# Autodesk Inventor assembly: outerHorn slider
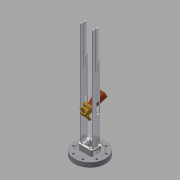
[picture p0: Inventor's stored thumbnail of the model, 180x180]
Saved by Autodesk Inventor 2015 SP1 (Build 190203100, 203)
## iProperties
Created: 2016-04-08
Part Number: outerHorn slider
Document SubType Name: Assembly
Designer: jad211
Author: jad211
## Documents named in this file (7)
- C:\ColdMatter\CADFiles\EDM Machine\Detection Region\Microwave Horn Assembly\outerHorn slider.iam
- C:\ColdMatter\CADFiles\EDM Machine\Detection Region\Microwave Horn Assembly\Horn with Flange.iam
- C:\ColdMatter\CADFiles\EDM Machine\Detection Region\Microwave Horn Assembly\Horn support.ipt
- C:\ColdMatter\CADFiles\EDM Machine\Pumping Region\coaxToWaveguidWG18.ipt
- C:\ColdMatter\CADFiles\EDM Machine\Detection Region\Microwave Horn Assembly\rod.ipt
- C:\ColdMatter\CADFiles\EDM Machine\Detection Region\Microwave Horn Assembly\DN63CF blank With Holes.ipt
- C:\ColdMatter\CADFiles\EDM Machine\Detection Region\Microwave Horn Assembly\supportHolder.ipt
## Components (10 placed, 6 different names)
1. Horn with Flange:1 [sub-assembly] — Mate:4, Mate:5, Flush:1, Mate:26, Mate:27, Mate:28, Mate:29, Mate:30, Mate:31, Mate:32
2. Horn support:1 — Flush:2, Mate:7, Mate:25, Mate:34
3. Horn support:2 — Flush:2, Mate:9, Flush:4, Mate:12, Mate:20, Mate:21, Angle:1, Mate:33, Mate:35
4. coaxToWaveguidWG18:1 — Mate:4, Mate:5, Flush:1
5. rod:1 — Mate:7
6. rod:2 — Mate:30, Mate:31, Mate:32
7. rod:4 — Mate:9, Flush:4, Mate:26
8. DN63CF blank With Holes:1 — Mate:12, Mate:17, Mate:18, Mate:19, Mate:21, Flush:5
9. rod:5 — Mate:28, Mate:29, Tangent:1
10. supportHolder:1 — Mate:17, Mate:18, Mate:19, Mate:25, Mate:34, Mate:35
## Relationships (27: Mate 21, Flush 4, Angle 1, Tangent 1)
- Mate:4: Horn with Flange:1 ↔ coaxToWaveguidWG18:1
- Mate:5: Horn with Flange:1 ↔ coaxToWaveguidWG18:1
- Flush:1: Horn with Flange:1 ↔ coaxToWaveguidWG18:1
- Flush:2: Horn support:1 ↔ Horn support:2
- Mate:7: Horn support:1 ↔ rod:1
- Mate:9: Horn support:2 ↔ rod:4
- Flush:4: Horn support:2 ↔ rod:4
- Mate:12: Horn support:2 ↔ DN63CF blank With Holes:1
- Mate:17: DN63CF blank With Holes:1 ↔ supportHolder:1
- Mate:18: DN63CF blank With Holes:1 ↔ supportHolder:1
- Mate:19: DN63CF blank With Holes:1 ↔ supportHolder:1
- Mate:20: Horn support:2
- Mate:21: Horn support:2 ↔ DN63CF blank With Holes:1
- Mate:25: Horn support:1 ↔ supportHolder:1
- Mate:26: Horn with Flange:1 ↔ rod:4
- Flush:5: DN63CF blank With Holes:1
- Mate:27: Horn with Flange:1
- Mate:28: Horn with Flange:1 ↔ rod:5
- Mate:29: Horn with Flange:1 ↔ rod:5
- Mate:30: Horn with Flange:1 ↔ rod:2
- Mate:31: Horn with Flange:1 ↔ rod:2
- Mate:32: Horn with Flange:1 ↔ rod:2
- Angle:1 (0 deg): Horn support:2
- Tangent:1: rod:5
- Mate:33 (0.025 mm): Horn support:2
- Mate:34: Horn support:1 ↔ supportHolder:1
- Mate:35: Horn support:2 ↔ supportHolder:1
